# Autodesk Inventor assembly: F1 Assembly
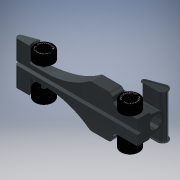
[picture p0: Inventor's stored thumbnail of the model, 180x180]
Saved by Autodesk Inventor 2019 (Build 230136000, 136)
## iProperties
Created: 2019-03-01
Part Number: F1 Assembly
Document SubType Name: Assembly
Designer: Raj
Author: Raj
## Documents named in this file (5)
- Y:\CADD\STUDENT WORK\5210537\TRACK B\02-C06\6 F1 CAR  (MINI PROJECT)\F1 Assembly.iam
- Y:\CADD\STUDENT WORK\5210537\TRACK B\02-C06\6 F1 CAR  (MINI PROJECT)\BODY.ipt
- Y:\CADD\STUDENT WORK\5210537\TRACK B\02-C06\6 F1 CAR  (MINI PROJECT)\Axle.ipt
- Y:\CADD\STUDENT WORK\5210537\TRACK B\02-C06\6 F1 CAR  (MINI PROJECT)\Wheel.ipt
- Y:\CADD\STUDENT WORK\5210537\TRACK B\02-C06\6 F1 CAR  (MINI PROJECT)\Retaining Ring.ipt
## Components (9 placed, 4 different names)
1. BODY:1 — Mate:1, Mate:4, Mate:5, Mate:6, Mate:7, Mate:10, Mate:12
2. Axle:1 — Mate:1, Mate:2, Mate:3, Mate:15, Mate:16
3. Axle:2 — Mate:7, Mate:8, Mate:9, Mate:11, Mate:13, Mate:14
4. Wheel:1 — Mate:2, Mate:3, Mate:4
5. Wheel:2 — Mate:5, Mate:6
6. Wheel:3 — Mate:8, Mate:9, Mate:10
7. Wheel:4 — Mate:11, Mate:12
8. Retaining Ring:2 — Mate:15, Mate:16
9. Retaining Ring:4 — Mate:13, Mate:14
## Relationships (16: Mate 16)
- Mate:1: BODY:1 ↔ Axle:1
- Mate:2: Axle:1 ↔ Wheel:1
- Mate:3: Axle:1 ↔ Wheel:1
- Mate:4: BODY:1 ↔ Wheel:1
- Mate:5: BODY:1 ↔ Wheel:2
- Mate:6: BODY:1 ↔ Wheel:2
- Mate:7: BODY:1 ↔ Axle:2
- Mate:8: Axle:2 ↔ Wheel:3
- Mate:9: Axle:2 ↔ Wheel:3
- Mate:10: BODY:1 ↔ Wheel:3
- Mate:11: Axle:2 ↔ Wheel:4
- Mate:12: BODY:1 ↔ Wheel:4
- Mate:13: Axle:2 ↔ Retaining Ring:4
- Mate:14: Axle:2 ↔ Retaining Ring:4
- Mate:15: Axle:1 ↔ Retaining Ring:2
- Mate:16: Axle:1 ↔ Retaining Ring:2
